# Autodesk Inventor assembly: ABD_Version 1.0
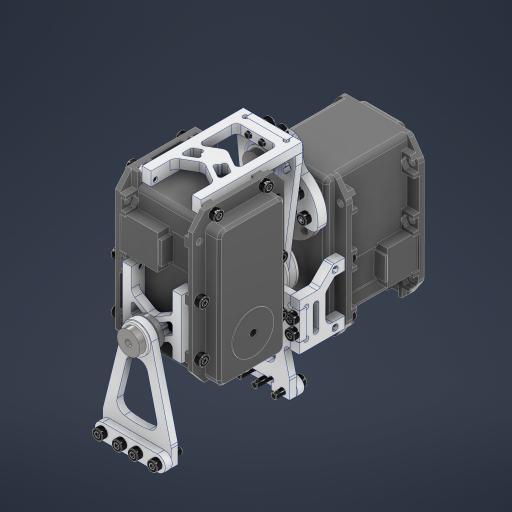
[picture p0: Inventor's stored thumbnail of the model, 512x512]
Saved by Autodesk Inventor 2024 (Build 280153000, 153)
## iProperties
Created: 2024-01-25
Part Number: ABD_Version 1.0
Document SubType Name: Assembly
Designer: ASUS
Author: ASUS
## Documents named in this file (11)
- C:\Users\ASUS\Desktop\Anti_Backlash_Structure_OP\v2_Frame\ABD_V2_Right_OP.iam
- C:\Users\ASUS\Desktop\Anti_Backlash_Structure_OP\v2_Frame\ABD_MX_64_Roll_Fixation_Set.iam
- C:\Users\ASUS\Desktop\Anti_Backlash_Structure_OP\v2_Frame\Roll_Fixation_Set.iam
- C:\Users\ASUS\Desktop\Anti_Backlash_Structure_OP\v2_Frame\ABD_MX_64_Slider_Fixation_Set_Left2Horn.iam
- C:\Users\ASUS\Desktop\Anti_Backlash_Structure_OP\MISUMI\C-WSSA12-4-2.ipt
- C:\Users\ASUS\Desktop\Anti_Backlash_Structure_OP\MISUMI\TT-0612-10.ipt
- C:\Users\ASUS\Desktop\Anti_Backlash_Structure_OP\MISUMI\LED-0606.ipt
- C:\Users\ASUS\Desktop\Anti_Backlash_Structure_OP\v3_Frame\Ubber_Washer_1.5mm.ipt
- C:\Users\ASUS\Desktop\Anti_Backlash_Structure_OP\MISUMI\TT-0612-5.ipt
- C:\Users\ASUS\Desktop\Anti_Backlash_Structure_OP\MISUMI\DBB4-8-5.ipt
- C:\Users\ASUS\Desktop\Anti_Backlash_Structure_OP\v3_Frame\ABD_Slider_Set_v3.iam
## Components (10 placed, 10 different names)
1. ABD_MX_64_Roll_Fixation_Set:1 [sub-assembly]
2. Roll_Fixation_Set:1 [sub-assembly] — 삽입:11
3. ABD_MX_64_Slider_Fixation_Set_Left2Horn:1 [sub-assembly] — 메이트:7, 메이트:8
4. C-WSSA12-4-2:1
5. TT-0612-10:1 — 삽입:10
6. LED-0606:1 — 메이트:7, 메이트:8
7. Ubber_Washer_1.5mm:1
8. TT-0612-5:1
9. DBB4-8-5:1
10. ABD_Slider_Set_v3:1 [sub-assembly] — 삽입:10, 삽입:11
## Relationships (13: Insert 8, Mate 5)
- [Insert]: ABD_MX_64_Roll_Fixation_Set:1 ↔ Roll_Fixation_Set:1
- [Mate]: ABD_MX_64_Roll_Fixation_Set:1 ↔ ABD_MX_64_Slider_Fixation_Set_Left2Horn:1
- [Mate]: ABD_MX_64_Roll_Fixation_Set:1 ↔ ABD_MX_64_Slider_Fixation_Set_Left2Horn:1
- [Mate] (0.05 mm): ABD_MX_64_Roll_Fixation_Set:1 ↔ ABD_MX_64_Slider_Fixation_Set_Left2Horn:1
- [Insert]: C-WSSA12-4-2:1 ↔ TT-0612-10:1
- [Insert]: C-WSSA12-4-2:1 ↔ LED-0606:1
- [Insert]: LED-0606:1 ↔ Ubber_Washer_1.5mm:1
- [Insert]: Ubber_Washer_1.5mm:1 ↔ TT-0612-5:1
- [Insert]: TT-0612-5:1 ↔ DBB4-8-5:1
- 메이트:7 [Mate]: ABD_MX_64_Slider_Fixation_Set_Left2Horn:1 ↔ LED-0606:1
- 삽입:10 [Insert]: TT-0612-10:1 ↔ ABD_Slider_Set_v3:1
- 삽입:11 [Insert] (-0.06 mm): Roll_Fixation_Set:1 ↔ ABD_Slider_Set_v3:1
- 메이트:8 [Mate] (0.025 mm): ABD_MX_64_Slider_Fixation_Set_Left2Horn:1 ↔ LED-0606:1
## Named parameters: d191_d198 = 0 mm, d192_d199 = 0 mm, d193_d200 = 0.05 mm
